# Autodesk Inventor assembly: R-wing
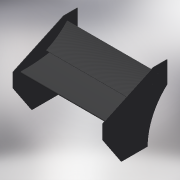
[picture p0: Inventor's stored thumbnail of the model, 180x180]
Saved by Autodesk Inventor 2018.2 (Build 222227000, 227)
## iProperties
Created: 2017-11-02
Part Number: R-wing
Material: 一般
Document SubType Name: Assembly
Designer: kuwano
Author: kuwano
## Documents named in this file (6)
- D:\kuwano\Documents\Inventor\KITformula\AeroCAD2018\CAD\Inventor\Aero Parts\R-wing\type6\R-wing.iam
- D:\kuwano\Documents\Inventor\KITformula\AeroCAD2018\CAD\Inventor\Aero Parts\R-wing\type6\parts\element_r_1.ipt
- D:\kuwano\Documents\Inventor\KITformula\AeroCAD2018\CAD\Inventor\Aero Parts\R-wing\type6\parts\end_plate.ipt
- D:\kuwano\Documents\Inventor\KITformula\AeroCAD2018\CAD\Inventor\Aero Parts\R-wing\type6\parts\end_plate_MIR.ipt
- D:\kuwano\Documents\Inventor\KITformula\AeroCAD2018\CAD\Inventor\Aero Parts\R-wing\type6\parts\cover_re.ipt
- D:\kuwano\Documents\Inventor\KITformula\AeroCAD2018\CAD\Inventor\Aero Parts\R-wing\type6\parts\element_clip.ipt
## Components (8 placed, 5 different names)
1. element_r_1:1 — フラッシュ:1, メイト:1, メイト:2, メイト:6, メイト:8, メイト:12, メイト:16, メイト:22, メイト:24, メイト:28, メイト:30
2. end_plate:1 — フラッシュ:3, フラッシュ:4, メイト:2, フラッシュ:6, メイト:13, メイト:17, メイト:29
3. end_plate_MIR:1 — フラッシュ:3, フラッシュ:4, メイト:1, メイト:7, メイト:9, メイト:23
4. cover_re:1 — フラッシュ:5
5. element_clip:2 — メイト:6, メイト:7, メイト:8, メイト:9
6. element_clip:4 — メイト:12, メイト:13, メイト:16, メイト:17
7. element_clip:6 — メイト:22, メイト:23, メイト:24
8. element_clip:8 — メイト:28, メイト:29, メイト:30
## Relationships (21: Mate 16, Flush 5)
- フラッシュ:1 [Flush]: element_r_1:1
- フラッシュ:3 [Flush]: end_plate:1 ↔ end_plate_MIR:1
- フラッシュ:4 [Flush]: end_plate:1 ↔ end_plate_MIR:1
- メイト:1 [Mate]: element_r_1:1 ↔ end_plate_MIR:1
- メイト:2 [Mate]: element_r_1:1 ↔ end_plate:1
- フラッシュ:5 [Flush]: cover_re:1
- メイト:6 [Mate]: element_r_1:1 ↔ element_clip:2
- メイト:7 [Mate]: end_plate_MIR:1 ↔ element_clip:2
- メイト:8 [Mate]: element_r_1:1 ↔ element_clip:2
- メイト:9 [Mate]: end_plate_MIR:1 ↔ element_clip:2
- フラッシュ:6 [Flush]: end_plate:1
- メイト:12 [Mate]: element_r_1:1 ↔ element_clip:4
- メイト:13 [Mate]: end_plate:1 ↔ element_clip:4
- メイト:16 [Mate]: element_r_1:1 ↔ element_clip:4
- メイト:17 [Mate]: end_plate:1 ↔ element_clip:4
- メイト:22 [Mate]: element_r_1:1 ↔ element_clip:6
- メイト:23 [Mate]: end_plate_MIR:1 ↔ element_clip:6
- メイト:24 [Mate]: element_r_1:1 ↔ element_clip:6
- メイト:28 [Mate]: element_r_1:1 ↔ element_clip:8
- メイト:29 [Mate]: end_plate:1 ↔ element_clip:8
- メイト:30 [Mate]: element_r_1:1 ↔ element_clip:8
